# Autodesk Inventor assembly: Final submission assembly
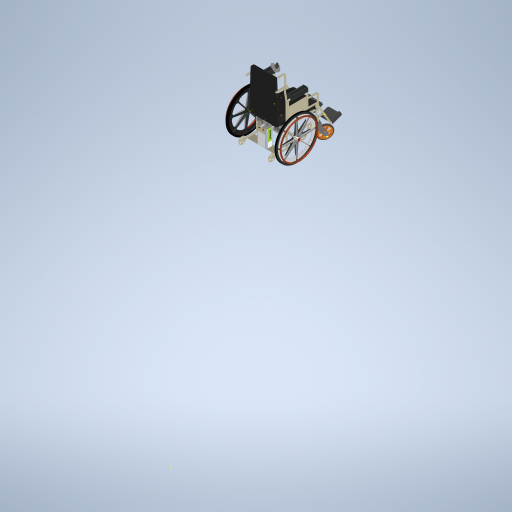
[picture p0: Inventor's stored thumbnail of the model, 512x512]
Saved by Autodesk Inventor 2023 (Build 270158000, 158)
## iProperties
Created: 2023-11-16
Part Number: Final submission assembly
Document SubType Name: Assembly
Designer: Raghav
Author: Raghav
## Documents named in this file (16)
- C:\Users\Dell\OneDrive - iitgn.ac.in\Sem_1\ES-101\Final submission assembly.iam
- C:\Users\Dell\OneDrive - iitgn.ac.in\Sem_1\ES-101\Course Project\Side frame model\Side frame.ipt
- C:\Users\Dell\OneDrive - iitgn.ac.in\Sem_1\ES-101\Course Project\Final assembly\Rear wheel.ipt
- C:\Users\Dell\OneDrive - iitgn.ac.in\Sem_1\ES-101\Course Project\Final assembly\Motor.ipt
- C:\Users\Dell\OneDrive - iitgn.ac.in\Sem_1\ES-101\Course Project\Final assembly\battery eg 26.ipt
- C:\Users\Dell\OneDrive - iitgn.ac.in\Sem_1\ES-101\Course Project\Final assembly\foot rest EG26.ipt
- C:\Users\Dell\OneDrive - iitgn.ac.in\Sem_1\ES-101\Course Project\Final assembly\Castorfork.ipt
- C:\Users\Dell\OneDrive - iitgn.ac.in\Sem_1\ES-101\Course Project\Final assembly\zfront wheel.ipt
- C:\Users\Dell\OneDrive - iitgn.ac.in\Sem_1\ES-101\Course Project\Parts for assembly\Anti tip wheels.ipt
- C:\Users\Dell\OneDrive - iitgn.ac.in\Sem_1\ES-101\Course Project\Final assembly\arm rest final 1.ipt
- C:\Users\Dell\OneDrive - iitgn.ac.in\Sem_1\ES-101\Course Project\Brakes\G26_P999999[4].ipt
- C:\Users\Dell\OneDrive - iitgn.ac.in\Sem_1\ES-101\Course Project\Brakes\G26_P999999[4L].ipt
- C:\Users\Dell\OneDrive - iitgn.ac.in\Sem_1\ES-101\Course Project\Final assembly\seatfinal.ipt
- C:\Users\Dell\OneDrive - iitgn.ac.in\Sem_1\ES-101\Course Project\Final assembly\backrest wheelchair EG26.ipt
- C:\Users\Dell\OneDrive - iitgn.ac.in\Sem_1\ES-101\Course Project\Final assembly\Joystick base.ipt
- C:\Users\Dell\OneDrive - iitgn.ac.in\Sem_1\ES-101\Course Project\Final assembly\Joystick upper.ipt
## Components (22 placed, 15 different names)
1. Side frame:1 — Rotational:1, Rotational:2, Rotational:3, Rotational:4, Rigid:1, Rotational:5, Rotational:6, Mate:1, Mate:2, Rotational:11, Rotational:12, Rigid:2, Rigid:3, Mate:3, Rigid:4, Mate:4, Rigid:5, Rigid:6
2. Rear wheel:1 — Rotational:5, Rotational:7
3. Rear wheel:2 — Rotational:6, Rotational:8
4. Motor:1 — Rotational:7, Mate:1
5. Motor:2 — Rotational:8, Mate:2
6. battery eg 26:1 — Rigid:1
7. foot rest EG26:1 — Rotational:11
8. foot rest EG26:2 — Rotational:12
9. Castorfork:1 — Rotational:3, Rotational:9
10. Castorfork:2 — Rotational:4, Rotational:10
11. zfront wheel:1 — Rotational:10
12. zfront wheel:2 — Rotational:9
13. Anti tip wheels:1 — Rotational:2
14. Anti tip wheels:2 — Rotational:1
15. arm rest final 1:1 — Rigid:2, Rigid:8
16. arm rest final 1:2 — Rigid:3
17. G26_P999999[4]:1 — Mate:4, Rigid:5
18. G26_P999999[4L]:1 — Mate:3, Rigid:4
19. seatfinal:1 — Rigid:6, Rigid:7
20. backrest wheelchair EG26:1 — Rigid:7
21. Joystick base:1 — Rigid:8, Ball:1
22. Joystick upper:1 — Ball:1
## Relationships (25: RevoluteJoint 12, WeldJoint 8, Mate 4, BallJoint 1)
- Rotational:1 [RevoluteJoint]: Side frame:1 ↔ Anti tip wheels:2
- Rotational:2 [RevoluteJoint]: Side frame:1 ↔ Anti tip wheels:1
- Rotational:3 [RevoluteJoint]: Side frame:1 ↔ Castorfork:1
- Rotational:4 [RevoluteJoint]: Side frame:1 ↔ Castorfork:2
- Rigid:1 [WeldJoint]: Side frame:1 ↔ battery eg 26:1
- Rotational:5 [RevoluteJoint]: Side frame:1 ↔ Rear wheel:1
- Rotational:6 [RevoluteJoint]: Side frame:1 ↔ Rear wheel:2
- Rotational:7 [RevoluteJoint]: Rear wheel:1 ↔ Motor:1
- Mate:1: Side frame:1 ↔ Motor:1
- Rotational:8 [RevoluteJoint]: Rear wheel:2 ↔ Motor:2
- Mate:2: Side frame:1 ↔ Motor:2
- Rotational:9 [RevoluteJoint]: Castorfork:1 ↔ zfront wheel:2
- Rotational:10 [RevoluteJoint]: Castorfork:2 ↔ zfront wheel:1
- Rotational:11 [RevoluteJoint]: Side frame:1 ↔ foot rest EG26:1
- Rotational:12 [RevoluteJoint]: Side frame:1 ↔ foot rest EG26:2
- Rigid:2 [WeldJoint]: Side frame:1 ↔ arm rest final 1:1
- Rigid:3 [WeldJoint]: Side frame:1 ↔ arm rest final 1:2
- Mate:3: Side frame:1 ↔ G26_P999999[4L]:1
- Rigid:4 [WeldJoint]: Side frame:1 ↔ G26_P999999[4L]:1
- Mate:4: Side frame:1 ↔ G26_P999999[4]:1
- Rigid:5 [WeldJoint]: Side frame:1 ↔ G26_P999999[4]:1
- Rigid:6 [WeldJoint]: Side frame:1 ↔ seatfinal:1
- Rigid:7 [WeldJoint]: seatfinal:1 ↔ backrest wheelchair EG26:1
- Rigid:8 [WeldJoint]: arm rest final 1:1 ↔ Joystick base:1
- Ball:1: Joystick base:1 ↔ Joystick upper:1
